# Autodesk Inventor assembly: beam_sub_asssem
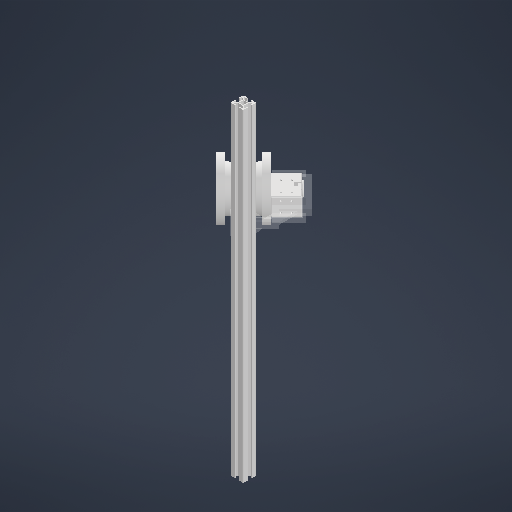
[picture p0: Inventor's stored thumbnail of the model, 512x512]
Saved by Autodesk Inventor 2026.2 (Build 302298010, 298A)
## iProperties
Created: 2026-02-11
Part Number: beam_sub_asssem
Document SubType Name: Assembly
Designer: Luke
Author: Luke
## Documents named in this file (3)
- C:\Users\Luke\OneDrive - Heriot-Watt University\Desktop\Robot Mech Sys\GroupProject\CAD\sub_assemblies\beam_sub_asssem.iam
- C:\Users\Luke\OneDrive - Heriot-Watt University\Desktop\Robot Mech Sys\GroupProject\CAD\parts\SIDE_BEAMS.ipt
- C:\Users\Luke\OneDrive - Heriot-Watt University\Desktop\Robot Mech Sys\GroupProject\CAD\sub_assemblies\motor_mount_sub_assem.iam
## Components (2 placed, 2 different names)
1. SIDE_BEAMS:1 — Mate:1, Mate:2, Mate:3
2. motor_mount_sub_assem:1 [sub-assembly] — Mate:1, Mate:2, Mate:3
## Relationships (3: Mate 3)
- Mate:1 (0.2 mm): SIDE_BEAMS:1 ↔ motor_mount_sub_assem:1
- Mate:2 (0.2 mm): SIDE_BEAMS:1 ↔ motor_mount_sub_assem:1
- Mate:3 (0.6 mm): SIDE_BEAMS:1 ↔ motor_mount_sub_assem:1
